# Autodesk Inventor assembly: FRC Arena 2013 (TEST VERSION) - top rung - 26x28 arpan version
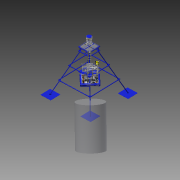
[picture p0: Inventor's stored thumbnail of the model, 180x180]
Saved by Autodesk Inventor 2013 (Build 170138000, 138)
## iProperties
Created: 2013-01-07
Part Number: FRC Arena 2013 (TEST VERSION) - top rung - 26x28 arpan version
Document SubType Name: Assembly
Designer: Phillip
Author: Phillip
## Documents named in this file (5)
- C:\Users\Arpan\Documents\GitHub\frc2013CAD\FIRST Arena 2013\FRC Arena 2013 (TEST VERSION) - top rung - 26x28 arpan version.iam
- C:\Users\Arpan\Documents\GitHub\frc2013CAD\FIRST Arena 2013\Arena\Arena Base.ipt
- C:\Users\Arpan\Documents\GitHub\frc2013CAD\FIRST Arena 2013\Pyramid\GE-13017.iam
- C:\Users\Arpan\Documents\GitHub\frc2013CAD\FIRST Arena 2013\Playing Configuration Constraint.ipt
- C:\Users\Arpan\Documents\GitHub\frc2013CAD\Robot Assembly - 6 wheel - toughbox mini - 26x28 screwed up by climber.iam
## Components (5 placed, 4 different names)
1. Arena Base:1 — Mate:2, Angle:1, Mate:3, Angle:2, Flush:3, Mate:41, Mate:42
2. GE-13017:1 [sub-assembly]
3. Robot Assembly - 6 wheel - toughbox mini - 26x28 screwed up by climber:1 [sub-assembly] — Mate:41, Mate:42, Tangent:9, Tangent:10
4. Playing Configuration Constraint:1
5. Playing Configuration Constraint:2 — Tangent:9, Tangent:10
## Relationships (11: Mate 4, Flush 3, Angle 2, Tangent 2)
- Mate:2: Arena Base:1
- Angle:1 (0 deg): Arena Base:1
- Flush:1 (2743.2 mm)
- Mate:3: Arena Base:1
- Angle:2 (0 deg): Arena Base:1
- Flush:2 (-2743.2 mm)
- Flush:3: Arena Base:1
- Mate:41 (1524 mm): Arena Base:1 ↔ Robot Assembly - 6 wheel - toughbox mini - 26x28 screwed up by climber:1
- Mate:42 (1524 mm): Arena Base:1 ↔ Robot Assembly - 6 wheel - toughbox mini - 26x28 screwed up by climber:1
- Tangent:9: Robot Assembly - 6 wheel - toughbox mini - 26x28 screwed up by climber:1 ↔ Playing Configuration Constraint:2
- Tangent:10: Robot Assembly - 6 wheel - toughbox mini - 26x28 screwed up by climber:1 ↔ Playing Configuration Constraint:2
